# Autodesk Inventor assembly: 組合檔
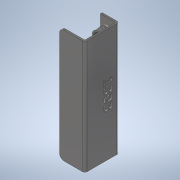
[picture p0: Inventor's stored thumbnail of the model, 180x180]
Saved by Autodesk Inventor 2020 (Build 240168000, 168)
## iProperties
Created: 2015-11-28
Part Number: 組合檔
Document SubType Name: Assembly
Designer: 設計製圖
Author: 設計製圖
## Documents named in this file (14)
- D:\資料庫\設計-3D Project\【May club 】\得利卡-車頂燈架\模型、圖面\短-車頂燈架-組合(#11.02)- 組合件2.iam
- D:\資料庫\設計-3D Project\【 鐵蹄 】\------鐵蹄工廠素材------ -\拉帽-M8.ipt
- D:\資料庫\設計-3D Project\材料庫\【螺絲】\止付螺絲\止付螺絲-M8-20.ipt
- D:\資料庫\設計-3D Project\【May club 】\得利卡-車頂燈架\模型、圖面\車身圖.ipt
- D:\資料庫\設計-3D Project\【May club 】\得利卡-車頂燈架\模型、圖面\吊架組件-ㄇ槽(#11.02).ipt
- D:\資料庫\設計-3D Project\【May club 】\得利卡-車頂燈架\模型、圖面\焊接組件-2(#11.02).ipt
- D:\資料庫\設計-3D Project\【May club 】\得利卡-車頂燈架\模型、圖面\得利卡-車頂導水槽.ipt
- D:\資料庫\設計-3D Project\材料庫\螺帽\白鐵-六角螺帽-M6.ipt
- D:\資料庫\設計-3D Project\【May club 】\得利卡-車頂燈架\模型、圖面\吊架-短(L)(#11.02)_MIR.ipt
- D:\資料庫\設計-3D Project\材料庫\【螺絲】\外六角螺絲\白鐵-外六角  M6-20.ipt
- D:\資料庫\設計-3D Project\材料庫\【華司】\白鐵-平面華司-7-16-2t.ipt
- D:\資料庫\設計-3D Project\材料庫\【華司】\彈簧華司\白鐵-彈簧華司-6.ipt
- D:\資料庫\設計-3D Project\【May club 】\得利卡-車頂燈架\模型、圖面\短-車頂燈架-組合(#11.02)-生產圖面_21.11.26\製程筆記\封邊條 ( 平光黑 ) - 130L.ipt
- D:\資料庫\設計-3D Project\【May club 】\得利卡-車頂燈架\模型、圖面\短-車頂燈架-組合(#11.02)-生產圖面_21.11.26\製程筆記\背膠海綿eva 6T -  15W x 125L.ipt
## Components (15 placed, 13 different names)
1. 拉帽-M8:2 — 齊平:6, 貼合:15, 貼合:32, 貼合:38
2. 拉帽-M8:1 — 齊平:6, 貼合:15, 貼合:17, 貼合:31, 貼合:37
3. 白鐵-六角螺帽-M6:1 — 貼合:44, 貼合:45, 齊平:15, 貼合:46
4. 吊架組件-ㄇ槽(#11.02):1 — 貼合:17, 貼合:37, 貼合:38, 貼合:40, 齊平:14, 貼合:41
5. 焊接組件-2(#11.02):1 — 貼合:40, 齊平:14, 貼合:41, 貼合:44, 貼合:45, 齊平:15
6. 吊架-短(L)(#11.02)_MIR:1 — 貼合:47
7. 得利卡-車頂導水槽:1
8. 車身圖:1
9. 背膠海綿eva 6T -  15W x 125L:1
10. 白鐵-彈簧華司-6:1 — 貼合:49, 貼合:51, 貼合:52
11. 白鐵-平面華司-7-16-2t:1 — 貼合:48, 貼合:51
12. 白鐵-外六角  M6-20:1 — 貼合:46, 貼合:48, 貼合:49, 貼合:52
13. 封邊條 ( 平光黑 ) - 130L:1
14. 止付螺絲-M8-20:1 — 齊平:12, 貼合:31
15. 止付螺絲-M8-20:2 — 齊平:12, 貼合:32
## Relationships (20: Mate 16, Flush 4)
- 齊平:6 [Flush]: 拉帽-M8:2 ↔ 拉帽-M8:1
- 貼合:15 [Mate]: 拉帽-M8:2 ↔ 拉帽-M8:1
- 貼合:17 [Mate]: 拉帽-M8:1 ↔ 吊架組件-ㄇ槽(#11.02):1
- 齊平:12 [Flush]: 止付螺絲-M8-20:1 ↔ 止付螺絲-M8-20:2
- 貼合:31 [Mate]: 拉帽-M8:1 ↔ 止付螺絲-M8-20:1
- 貼合:32 [Mate]: 拉帽-M8:2 ↔ 止付螺絲-M8-20:2
- 貼合:37 [Mate]: 拉帽-M8:1 ↔ 吊架組件-ㄇ槽(#11.02):1
- 貼合:38 [Mate]: 拉帽-M8:2 ↔ 吊架組件-ㄇ槽(#11.02):1
- 貼合:40 [Mate]: 吊架組件-ㄇ槽(#11.02):1 ↔ 焊接組件-2(#11.02):1
- 齊平:14 [Flush]: 吊架組件-ㄇ槽(#11.02):1 ↔ 焊接組件-2(#11.02):1
- 貼合:41 [Mate]: 吊架組件-ㄇ槽(#11.02):1 ↔ 焊接組件-2(#11.02):1
- 貼合:44 [Mate]: 白鐵-六角螺帽-M6:1 ↔ 焊接組件-2(#11.02):1
- 貼合:45 [Mate]: 白鐵-六角螺帽-M6:1 ↔ 焊接組件-2(#11.02):1
- 齊平:15 [Flush]: 白鐵-六角螺帽-M6:1 ↔ 焊接組件-2(#11.02):1
- 貼合:46 [Mate]: 白鐵-六角螺帽-M6:1 ↔ 白鐵-外六角  M6-20:1
- 貼合:47 [Mate] (150 mm): 吊架-短(L)(#11.02)_MIR:1
- 貼合:48 [Mate]: 白鐵-平面華司-7-16-2t:1 ↔ 白鐵-外六角  M6-20:1
- 貼合:49 [Mate]: 白鐵-彈簧華司-6:1 ↔ 白鐵-外六角  M6-20:1
- 貼合:51 [Mate]: 白鐵-彈簧華司-6:1 ↔ 白鐵-平面華司-7-16-2t:1
- 貼合:52 [Mate]: 白鐵-彈簧華司-6:1 ↔ 白鐵-外六角  M6-20:1
